# Autodesk Inventor assembly: Wheel
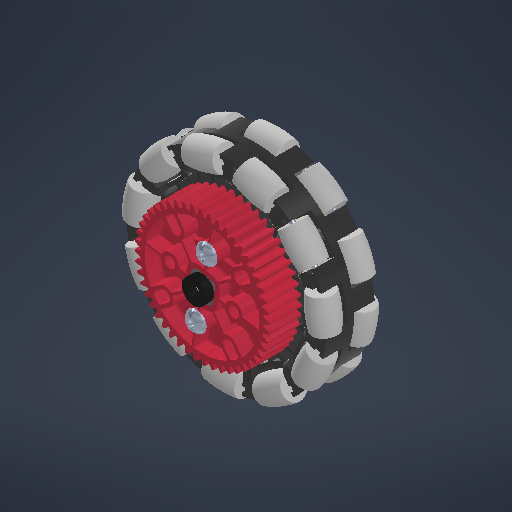
[picture p0: Inventor's stored thumbnail of the model, 512x512]
Saved by Autodesk Inventor 2026.1 (Build 301233000, 233)
## iProperties
Created: 2025-08-03
Part Number: Wheel
Document SubType Name: Assembly
Designer: roejo
Author: roejo
## Documents named in this file (14)
- C:\Users\roejo\OneDrive\Documents\3284b-highlander-cad\Robots\Highlander\SubAssemblies\Wheel.iam
- C:\Users\roejo\OneDrive\Documents\3284b-highlander-cad\Library\VEX-CAD-Inventor-1.4.2\Motion\Wheels\Omni Wheel.iam
- C:\Users\roejo\OneDrive\Documents\3284b-highlander-cad\Library\Custom Parts\HS 48T Gear, No Insert, Lathe.iam
- C:\Users\roejo\OneDrive\Documents\3284b-highlander-cad\Library\VEX-CAD-Inventor-1.4.2\Motion\Gears\HS Gear.iam
- C:\Users\roejo\OneDrive\Documents\3284b-highlander-cad\Library\VEX-CAD-Inventor-1.4.2\Motion\Spacers\Washer Teflon\TWasher .375 OD x .06250.ipt
- C:\Users\roejo\OneDrive\Documents\3284b-highlander-cad\Library\VEX-CAD-Inventor-1.4.2\Motion\Spacers\Washer Teflon.ipt
- C:\Users\roejo\OneDrive\Documents\3284b-highlander-cad\Library\VEX-CAD-Inventor-1.4.2\Motion\Spacers\Spacer Nylon .375 OD\NSpacer .375 OD x .125.ipt
- C:\Users\roejo\OneDrive\Documents\3284b-highlander-cad\Library\VEX-CAD-Inventor-1.4.2\Motion\Spacers\Spacer Nylon .375 OD.ipt
- C:\Users\roejo\OneDrive\Documents\3284b-highlander-cad\Library\VEX-CAD-Inventor-1.4.2\Structure\Hardware\alu_nylock.ipt
- C:\Users\roejo\OneDrive\Documents\3284b-highlander-cad\Library\VEX-CAD-Inventor-1.4.2\Structure\Standoff\Standoff .50.ipt
- C:\Users\roejo\OneDrive\Documents\3284b-highlander-cad\Library\VEX-CAD-Inventor-1.4.2\Structure\Standoff.ipt
- C:\Users\roejo\OneDrive\Documents\3284b-highlander-cad\Library\VEX-CAD-Inventor-1.4.2\Structure\Hardware\Screw Steel - Star.ipt
- C:\Users\roejo\OneDrive\Documents\3284b-highlander-cad\Library\VEX-CAD-Inventor-1.4.2\Structure\Hardware\Screw Steel - Star\SScrew Star Smooth 1.250.ipt
- C:\Users\roejo\OneDrive\Documents\3284b-highlander-cad\Library\VEX-CAD-Inventor-1.4.2\Motion\Wheels\Omni Wheel\3.25 Omni AS, No Insert.iam
## Components (10 placed, 7 different names)
1. HS 48T Gear, No Insert, Lathe:1 [sub-assembly] — Insert:3, Insert:11, Insert:13, Insert:14, Insert:15
2. NSpacer .375 OD x .125:1 — Insert:3
3. TWasher .375 OD x .06250:1 — Insert:5, Insert:18
4. alu_nylock:1 — Insert:5, Insert:6
5. Standoff .50:1 — Insert:6
6. alu_nylock:4 — Insert:17
7. SScrew Star Smooth 1.250:4 — Insert:11
8. alu_nylock:5 — Insert:16
9. SScrew Star Smooth 1.250:5 — Insert:13
10. 3.25 Omni AS, No Insert:1 [sub-assembly] — Insert:14, Insert:15, Insert:16, Insert:17, Insert:18
## Relationships (10: Insert 10)
- Insert:3: HS 48T Gear, No Insert, Lathe:1 ↔ NSpacer .375 OD x .125:1
- Insert:5: TWasher .375 OD x .06250:1 ↔ alu_nylock:1
- Insert:6: alu_nylock:1 ↔ Standoff .50:1
- Insert:11: HS 48T Gear, No Insert, Lathe:1 ↔ SScrew Star Smooth 1.250:4
- Insert:13: HS 48T Gear, No Insert, Lathe:1 ↔ SScrew Star Smooth 1.250:5
- Insert:14: HS 48T Gear, No Insert, Lathe:1 ↔ 3.25 Omni AS, No Insert:1
- Insert:15: HS 48T Gear, No Insert, Lathe:1 ↔ 3.25 Omni AS, No Insert:1
- Insert:16: alu_nylock:5 ↔ 3.25 Omni AS, No Insert:1
- Insert:17: alu_nylock:4 ↔ 3.25 Omni AS, No Insert:1
- Insert:18: TWasher .375 OD x .06250:1 ↔ 3.25 Omni AS, No Insert:1
